# Autodesk Inventor assembly: FrontGearboxAssembly
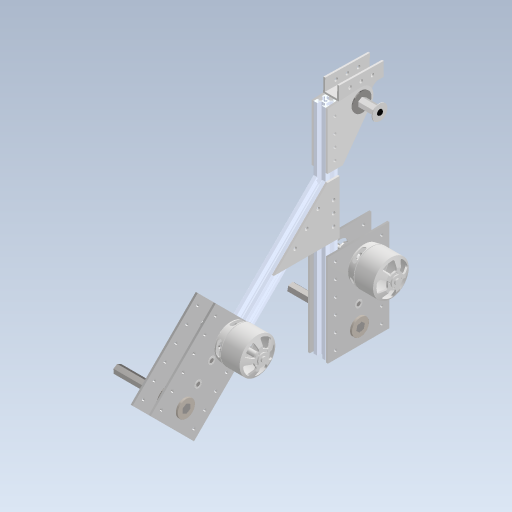
[picture p0: Inventor's stored thumbnail of the model, 512x512]
Saved by Autodesk Inventor 2023 (Build 270158000, 158)
## iProperties
Created: 2023-02-14
Part Number: FrontGearboxAssembly
Document SubType Name: Assembly
Designer: Dave
Author: Dave
## Documents named in this file (7)
- C:\Users\Dave\Documents\GitHub\BehrendURCMechanical\CAD\Chassis\GearBox\Final Gears and Assemblies\FrontGearboxAssembly.iam
- C:\Users\Dave\Documents\GitHub\BehrendURCMechanical\CAD\Chassis\GearBox\Final Gears and Assemblies\Gearbox Assembly.iam
- C:\Users\Dave\Documents\GitHub\BehrendURCMechanical\CAD\Chassis\20 Profile\CH-1-01-20 Channel 0.32 Angle.ipt
- C:\Users\Dave\Documents\GitHub\BehrendURCMechanical\CAD\Chassis\20 Profile\CH-1-01-20 Channel 0.362m.ipt
- C:\Users\Dave\Documents\GitHub\BehrendURCMechanical\CAD\Chassis\CH-1-01-FrontKneeJoint.ipt
- C:\Users\Dave\Documents\GitHub\BehrendURCMechanical\CAD\Chassis\HipJoint.iam
- C:\Users\Dave\Documents\GitHub\BehrendURCMechanical\CAD\Chassis\GearBox\Final Gears and Assemblies\CH-1-01-BearingBracket (2).ipt
## Components (7 placed, 6 different names)
1. Gearbox Assembly:1 [sub-assembly] — Angle:1, Flush:1, Angle:2, Flush:2, Mate:1, Flush:3
2. Gearbox Assembly:2 [sub-assembly] — Flush:1, Angle:2, Flush:5, Flush:10
3. CH-1-01-20 Channel 0.32 Angle:1 — Mate:2, Flush:4, Flush:5, Flush:8, Flush:10
4. CH-1-01-20 Channel 0.362m:1 — Flush:2, Mate:1, Flush:3, Mate:2, Flush:4, Flush:7, Mate:9, Flush:9, Mate:10, Mate:11
5. CH-1-01-FrontKneeJoint:1 — Flush:7, Mate:9, Flush:8
6. HipJoint:1 [sub-assembly] — Flush:9, Mate:10, Mate:11, Mate:12, Mate:13
7. CH-1-01-BearingBracket (2):1 — Mate:12, Mate:13
## Relationships (18: Flush 9, Mate 7, Angle 2)
- Angle:1 (90 deg): Gearbox Assembly:1
- Flush:1: Gearbox Assembly:1 ↔ Gearbox Assembly:2
- Angle:2 (-45 deg): Gearbox Assembly:1 ↔ Gearbox Assembly:2
- Flush:2: Gearbox Assembly:1 ↔ CH-1-01-20 Channel 0.362m:1
- Mate:1 (3.31 mm): Gearbox Assembly:1 ↔ CH-1-01-20 Channel 0.362m:1
- Flush:3 (2.6924 mm): Gearbox Assembly:1 ↔ CH-1-01-20 Channel 0.362m:1
- Mate:2: CH-1-01-20 Channel 0.32 Angle:1 ↔ CH-1-01-20 Channel 0.362m:1
- Flush:4: CH-1-01-20 Channel 0.32 Angle:1 ↔ CH-1-01-20 Channel 0.362m:1
- Flush:5: Gearbox Assembly:2 ↔ CH-1-01-20 Channel 0.32 Angle:1
- Flush:7: CH-1-01-20 Channel 0.362m:1 ↔ CH-1-01-FrontKneeJoint:1
- Mate:9: CH-1-01-20 Channel 0.362m:1 ↔ CH-1-01-FrontKneeJoint:1
- Flush:8: CH-1-01-20 Channel 0.32 Angle:1 ↔ CH-1-01-FrontKneeJoint:1
- Flush:9: CH-1-01-20 Channel 0.362m:1 ↔ HipJoint:1
- Mate:10: CH-1-01-20 Channel 0.362m:1 ↔ HipJoint:1
- Mate:11: CH-1-01-20 Channel 0.362m:1 ↔ HipJoint:1
- Mate:12: HipJoint:1 ↔ CH-1-01-BearingBracket (2):1
- Mate:13: HipJoint:1 ↔ CH-1-01-BearingBracket (2):1
- Flush:10 (-2.6924 mm): Gearbox Assembly:2 ↔ CH-1-01-20 Channel 0.32 Angle:1
